# Autodesk Inventor assembly: Cascade Pulley Block (WCP-0298)
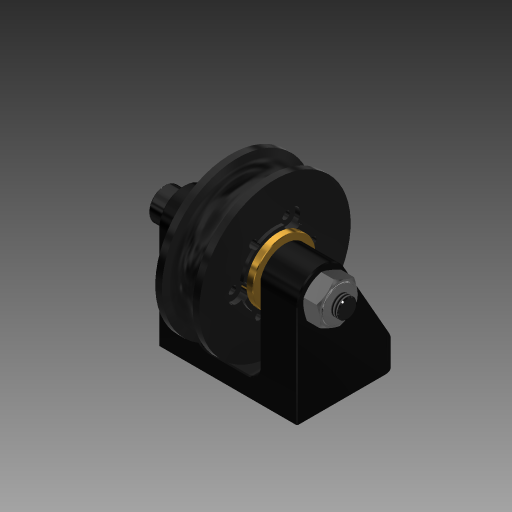
[picture p0: Inventor's stored thumbnail of the model, 512x512]
Saved by Autodesk Inventor 2023 (Build 270158000, 158)
## iProperties
Created: 2023-01-15
Part Number: Cascade Pulley Block (WCP-0298)
Document SubType Name: Assembly
Designer: Max Boord
Mass: 63.5166 g
Surface Area: 160.946 cm^2
Volume: 22.646 cm^3
Density: 2.80476 g/cm^3
Author: Max Boord
## iProperties of the stored document MemberDocs/xU3tbij54N0dk4bpbX2j5xmkeEf
Created: 2023-01-15
Part Number: Cascade Pulley Block (WCP-0298)
Document SubType Name: Assembly
Designer: Max Boord
Mass: 63.5166 g
Surface Area: 160.946 cm^2
Volume: 22.646 cm^3
Density: 2.80476 g/cm^3
Author: Max Boord
## iProperties of the stored document MemberDocs/xHnjutmj3N0mzab5oUacbvizwMc
Created: 2023-01-15
Part Number: Cascade Pulley Block (WCP-0298)
Document SubType Name: Assembly
Designer: Max Boord
Mass: 83.114 g
Surface Area: 133.642 cm^2
Volume: 25.0968 cm^3
Density: 3.31174 g/cm^3
Author: Max Boord
## iProperties of the stored document MemberDocs/xVoehj15mBcigi0ksDjhrpxdkQg
Created: 2023-01-15
Part Number: Cascade Pulley Block (WCP-0298)
Document SubType Name: Assembly
Designer: Max Boord
Mass: 63.5166 g
Surface Area: 160.946 cm^2
Volume: 22.646 cm^3
Density: 2.80476 g/cm^3
Author: Max Boord
## Documents named in this file (21)
- E:\Collaborative Robots\Collaborative Part Library\Elevators\GreyT Elevator Parts\Cascade Pulley Block (WCP-0298).iam
- E:\Collaborative Robots\Collaborative Part Library\Elevators\GreyT Elevator Parts\Cascade Pulley Block (WCP-0298).ipt
- E:\Collaborative Robots\Collaborative Part Library\Power Transfer\Belts and Pullies\WCP Polycord Pulley States.ipt
- E:\Collaborative Robots\Collaborative Part Library\Power Transfer\Bearings and Bushings\WCP 500 Hex Bushing.ipt
- E:\Collaborative Robots\Collaborative Part Library\Hardware\Spacers\Spacers & Standoffs\WCP Aluminum Standoff (No. 10 x 0.625Lg x 0.375OD).ipt
- E:\Collaborative Robots\Collaborative Part Library\Hardware\Spacers\Spacers & Standoffs.ipt
- E:\Collaborative Robots\Collaborative Part Library\Hardware\Fasteners\Machine Screws.ipt
- E:\Collaborative Robots\Collaborative Part Library\Hardware\Nuts and Threaded Blocks\Nuts\10-32 Pan Head Nylon locknut.ipt
- E:\Collaborative Robots\Collaborative Part Library\Hardware\Nuts and Threaded Blocks\Nuts.ipt
- E:\Collaborative Robots\Collaborative Part Library\Hardware\Fasteners\Machine Screws\10-32 UNFx1.625 Socket Head Cap Screw.ipt
- E:\Collaborative Robots\Collaborative Part Library\Elevators\GreyT Elevator Parts\0.625in LG x 1032 x 0.25in OD Round Standoff (McMaster Carr 93330A469).ipt
- E:\Collaborative Robots\Collaborative Part Library\Elevators\GreyT Elevator Parts\Custom Cascade Bearing Pulley.ipt
- E:\Collaborative Robots\Collaborative Part Library\Power Transfer\Bearings and Bushings\Bearings.ipt
- E:\Collaborative Robots\Collaborative Part Library\Power Transfer\Bearings and Bushings\Bearings\FR4.ipt
- E:\Collaborative Robots\Collaborative Part Library\Elevators\GreyT Elevator Parts\98126A647_18-8 Stainless Steel Ring Shim.ipt
- D:\Collaborative Robots\COTS Parts\Elevators\GreyT Elevator Parts\Cascade Pulley Block (WCP-0298).ipt
- D:\Collaborative Robots\COTS Parts\Power Transfer\Belts and Pullies\WCP Polycord Pulley States.ipt
- D:\Collaborative Robots\COTS Parts\Power Transfer\Bearings and Bushings\WCP 500 Hex Bushing.ipt
- D:\Collaborative Robots\COTS Parts\Hardware\Spacers\Spacers & Standoffs\WCP Aluminum Standoff (No. 10 x 0.625Lg x 0.375OD).ipt
- D:\Collaborative Robots\COTS Parts\Hardware\Nuts and Threaded Blocks\Nuts\10-32 Pan Head Nylon locknut.ipt
- D:\Collaborative Robots\COTS Parts\Hardware\Fasteners\Machine Screws\10-32 UNFx1.625 Socket Head Cap Screw.ipt
## Components (8 placed, 6 different names)
1. Cascade Pulley Block (WCP-0298):1 — Mate:2, Flush:1, Mate:8, Insert:5, Mate:9, Flush:2, Insert:6
2. WCP Polycord Pulley States:1 — Insert:1, Mate:1, Insert:2, Mate:2, Mate:7, Mate:10
3. WCP Polycord Pulley States:2 — Insert:1, Mate:1, Insert:3, Mate:10
4. WCP 500 Hex Bushing:1 — Insert:3, Mate:4
5. WCP 500 Hex Bushing:2 — Insert:2
6. WCP Aluminum Standoff (No. 10 x 0.625Lg x 0.375OD):1 — Mate:4, Flush:1, Mate:9
7. 10-32 UNFx1.625 Socket Head Cap Screw:1 — Insert:4, Insert:5, Insert:6
8. 10-32 Pan Head Nylon locknut:1 — Insert:4
## Relationships (15: Mate 7, Insert 6, Flush 2)
- Insert:1: WCP Polycord Pulley States:1 ↔ WCP Polycord Pulley States:2
- Mate:1: WCP Polycord Pulley States:1 ↔ WCP Polycord Pulley States:2
- Insert:2: WCP Polycord Pulley States:1 ↔ WCP 500 Hex Bushing:2
- Insert:3: WCP Polycord Pulley States:2 ↔ WCP 500 Hex Bushing:1
- Mate:2: Cascade Pulley Block (WCP-0298):1 ↔ WCP Polycord Pulley States:1
- Mate:4: WCP 500 Hex Bushing:1 ↔ WCP Aluminum Standoff (No. 10 x 0.625Lg x 0.375OD):1
- Flush:1: Cascade Pulley Block (WCP-0298):1 ↔ WCP Aluminum Standoff (No. 10 x 0.625Lg x 0.375OD):1
- Mate:7: WCP Polycord Pulley States:1
- Mate:8: Cascade Pulley Block (WCP-0298):1
- Insert:4 (34.925 mm): 10-32 UNFx1.625 Socket Head Cap Screw:1 ↔ 10-32 Pan Head Nylon locknut:1
- Insert:5: Cascade Pulley Block (WCP-0298):1 ↔ 10-32 UNFx1.625 Socket Head Cap Screw:1
- Mate:9: Cascade Pulley Block (WCP-0298):1 ↔ WCP Aluminum Standoff (No. 10 x 0.625Lg x 0.375OD):1
- Flush:2: Cascade Pulley Block (WCP-0298):1
- Mate:10: WCP Polycord Pulley States:1 ↔ WCP Polycord Pulley States:2
- Insert:6: Cascade Pulley Block (WCP-0298):1 ↔ 10-32 UNFx1.625 Socket Head Cap Screw:1
